# Autodesk Inventor assembly: neverest 40 + mounts + pulley + compliant wheel
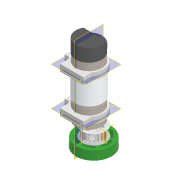
[picture p0: Inventor's stored thumbnail of the model, 180x180]
Saved by Autodesk Inventor 2020 (Build 240168000, 168)
## iProperties
Created: 2020-02-12
Part Number: neverest 40 + mounts + pulley + compliant wheel
Document SubType Name: Assembly
Designer: ball
Author: ball
## Documents named in this file (3)
- C:\FTC\FTC8863CAD\2019 Robot\Collection\neverest 40 + mounts + pulley + compliant wheel.iam
- C:\FTC\FTC8863CAD\2019 Robot\Collection\neverest 40 + mounts.iam
- C:\FTC\FTC8863CAD\2019 Robot\general robot componets\pulley .25 in + wheel.2.iam
## Components (2 placed, 2 different names)
1. neverest 40 + mounts:1 [sub-assembly] — Mate:1, Mate:2
2. pulley .25 in + wheel.2:1 [sub-assembly] — Mate:1, Mate:2
## Relationships (2: Mate 2)
- Mate:1: neverest 40 + mounts:1 ↔ pulley .25 in + wheel.2:1
- Mate:2: neverest 40 + mounts:1 ↔ pulley .25 in + wheel.2:1
